# Autodesk Inventor assembly: アーム ツインロッドアーム先端アセンブリ
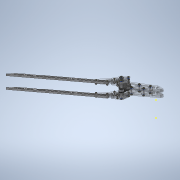
[picture p0: Inventor's stored thumbnail of the model, 180x180]
Saved by Autodesk Inventor 2020.2 (Build 242310000, 310)
## iProperties
Created: 2018-11-26
Part Number: アーム ツインロッドアーム先端アセンブリ
Material: 一般
Document SubType Name: Assembly
Designer: 雪村
Mass: 174.621 g
Surface Area: 858.198 cm^2
Volume: 87.2019 cm^3
Density: 2.00249 g/cm^3
Author: 雪村
## Documents named in this file (16)
- C:\Users\mozar\Desktop\院2年機大型\アーム ツインロッドアーム先端アセンブリ.iam
- C:\Users\mozar\Desktop\院2年機大型\アーム アーム先端根本ポリカパーツ.ipt
- C:\Users\mozar\Desktop\院2年機大型\アーム アーム先端根本ポリカパーツ(ミラー).ipt
- C:\Users\mozar\Desktop\院2年機大型\既製品\スペーサーm3-16　簡易筒型.ipt
- C:\Users\mozar\Desktop\院2年機大型\アーム ツインアーム先端押さえ.ipt
- C:\Users\mozar\Desktop\院2年機大型\既製品\ねじ\SB　M4 8mm なべネジ.ipt
- C:\Users\mozar\Desktop\院2年機大型\既製品\セットカラー　内径6.ipt
- C:\Users\mozar\Desktop\院2年機大型\アーム 中間節 先端中詰め.ipt
- C:\Users\mozar\Desktop\院2年機大型\既製品\スペーサーm3-60　簡易筒型　売ってない.ipt
- C:\Users\mozar\Desktop\院2年機大型\既製品\ねじ\SB　6mmなべネジ.ipt
- C:\Users\mozar\Desktop\院2年機大型\既製品\ねじ\ナイロンナットm3.ipt
- C:\Users\mozar\Desktop\院2年機大型\アーム アーム先端長め丹治type.ipt
- C:\Users\mozar\Desktop\院2年機大型\アーム ツインアーム先端 ポリカフリー部5t(ミラー).ipt
- C:\Users\mozar\Desktop\院2年機大型\アーム ツインアーム先端 ポリカフリー部5t.ipt
- C:\Users\mozar\Desktop\院2年機大型\既製品\オイレス　6-8-12　フランジ付き　（L=5）.ipt
- C:\Users\mozar\Desktop\院2年機大型\既製品\ねじ\SB　14mmなべネジ.ipt
## Components (60 placed, 15 different names)
1. アーム アーム先端根本ポリカパーツ:1 — 挿入:230, 挿入:231, 挿入:232, 挿入:233, 挿入:250, 挿入:251, 挿入:252, 挿入:253, メイト:10
2. アーム アーム先端根本ポリカパーツ(ミラー):1 — 挿入:246, 挿入:247, 挿入:248, 挿入:249, 挿入:259, メイト:8, メイト:9, 挿入:294
3. アーム ツインアーム先端押さえ:1 — 挿入:265, 挿入:266, 挿入:268, 挿入:269, 挿入:270
4. アーム ツインアーム先端押さえ:2 — 挿入:260, 挿入:261, 挿入:262, 挿入:271, 挿入:272, 挿入:273
5. スペーサーm3-16　簡易筒型:4 — 挿入:230
6. スペーサーm3-16　簡易筒型:5 — 挿入:231, 挿入:294
7. スペーサーm3-16　簡易筒型:6 — 挿入:232
8. スペーサーm3-16　簡易筒型:7 — 挿入:233
9. SB　M4 8mm なべネジ:6 — 挿入:248
10. SB　M4 8mm なべネジ:8 — 挿入:249
11. SB　M4 8mm なべネジ:9 — 挿入:252
12. SB　M4 8mm なべネジ:14 — 挿入:246
13. SB　M4 8mm なべネジ:17 — 挿入:247
14. SB　M4 8mm なべネジ:18 — 挿入:250
15. SB　M4 8mm なべネジ:19 — 挿入:251
16. SB　M4 8mm なべネジ:20 — 挿入:253
17. セットカラー　内径6:3 — 挿入:255
18. セットカラー　内径6:4 — 挿入:254, 挿入:257
19. セットカラー　内径6:5 — 挿入:256, 挿入:258
20. アーム 中間節 先端中詰め:1 — 挿入:254, 挿入:255, 挿入:256
21. アーム 中間節 先端中詰め:2 — 挿入:257, 挿入:258, 挿入:259, メイト:8
22. スペーサーm3-60　簡易筒型　売ってない:1 — 挿入:260, メイト:9, 挿入:266, メイト:10
23. スペーサーm3-60　簡易筒型　売ってない:2 — 挿入:261, 挿入:265, 挿入:307, 挿入:308
24. スペーサーm3-60　簡易筒型　売ってない:3 — 挿入:262
25. SB　6mmなべネジ:1 — 挿入:268
26. SB　6mmなべネジ:2 — 挿入:270
27. SB　6mmなべネジ:3 — 挿入:269
28. SB　6mmなべネジ:4 — 挿入:273
29. SB　6mmなべネジ:5 — 挿入:272
30. SB　6mmなべネジ:6 — 挿入:271
31. ナイロンナットm3:1 — 挿入:326
32. ナイロンナットm3:5 — 挿入:324
33. ナイロンナットm3:12 — 挿入:327
34. ナイロンナットm3:13 — 挿入:320
35. ナイロンナットm3:14 — 挿入:325
36. ナイロンナットm3:16 — 挿入:319
37. ナイロンナットm3:17 — 挿入:328
38. アーム アーム先端長め丹治type:1 — 挿入:303, 挿入:304
39. アーム アーム先端長め丹治type:2 — 挿入:305, 挿入:306
40. アーム ツインアーム先端 ポリカフリー部5t(ミラー):1 — 挿入:296, 挿入:299, 挿入:300, 挿入:314, 挿入:315, 挿入:316, 挿入:317, 挿入:318
41. アーム ツインアーム先端 ポリカフリー部5t:1 — 挿入:295, 挿入:299, 挿入:300, 挿入:303, 挿入:304, 挿入:319, 挿入:320, 挿入:321, 挿入:322, 挿入:323
42. アーム ツインアーム先端 ポリカフリー部5t(ミラー):2 — 挿入:297, 挿入:301, 挿入:302, 挿入:324, 挿入:325, 挿入:326, 挿入:327, 挿入:328
43. アーム ツインアーム先端 ポリカフリー部5t:2 — 挿入:298, 挿入:301, 挿入:302, 挿入:305, 挿入:306, 挿入:309, 挿入:310, 挿入:311, 挿入:312, 挿入:313
44. オイレス　6-8-12　フランジ付き　（L=5）:1 — 挿入:297
45. オイレス　6-8-12　フランジ付き　（L=5）:2 — 挿入:298, 挿入:308
46. オイレス　6-8-12　フランジ付き　（L=5）:3 — 挿入:296, 挿入:307
47. オイレス　6-8-12　フランジ付き　（L=5）:4 — 挿入:295
48. SB　14mmなべネジ:1 — 挿入:310
49. SB　14mmなべネジ:2 — 挿入:311
50. SB　14mmなべネジ:3 — 挿入:309
51. SB　14mmなべネジ:4 — 挿入:312
52. SB　14mmなべネジ:5 — 挿入:318
53. SB　14mmなべネジ:6 — 挿入:316
54. SB　14mmなべネジ:7 — 挿入:315
55. SB　14mmなべネジ:8 — 挿入:317
56. SB　14mmなべネジ:9 — 挿入:314
57. SB　14mmなべネジ:10 — 挿入:313
58. ナイロンナットm3:18 — 挿入:321
59. ナイロンナットm3:19 — 挿入:322
60. ナイロンナットm3:20 — 挿入:323
## Relationships (67: Insert 64, Mate 3)
- 挿入:230 [Insert]: アーム アーム先端根本ポリカパーツ:1 ↔ スペーサーm3-16　簡易筒型:4
- 挿入:231 [Insert]: アーム アーム先端根本ポリカパーツ:1 ↔ スペーサーm3-16　簡易筒型:5
- 挿入:232 [Insert]: アーム アーム先端根本ポリカパーツ:1 ↔ スペーサーm3-16　簡易筒型:6
- 挿入:233 [Insert]: アーム アーム先端根本ポリカパーツ:1 ↔ スペーサーm3-16　簡易筒型:7
- 挿入:246 [Insert]: アーム アーム先端根本ポリカパーツ(ミラー):1 ↔ SB　M4 8mm なべネジ:14
- 挿入:247 [Insert]: アーム アーム先端根本ポリカパーツ(ミラー):1 ↔ SB　M4 8mm なべネジ:17
- 挿入:248 [Insert]: アーム アーム先端根本ポリカパーツ(ミラー):1 ↔ SB　M4 8mm なべネジ:6
- 挿入:249 [Insert]: アーム アーム先端根本ポリカパーツ(ミラー):1 ↔ SB　M4 8mm なべネジ:8
- 挿入:250 [Insert]: アーム アーム先端根本ポリカパーツ:1 ↔ SB　M4 8mm なべネジ:18
- 挿入:251 [Insert]: アーム アーム先端根本ポリカパーツ:1 ↔ SB　M4 8mm なべネジ:19
- 挿入:252 [Insert]: アーム アーム先端根本ポリカパーツ:1 ↔ SB　M4 8mm なべネジ:9
- 挿入:253 [Insert]: アーム アーム先端根本ポリカパーツ:1 ↔ SB　M4 8mm なべネジ:20
- 挿入:254 [Insert]: セットカラー　内径6:4 ↔ アーム 中間節 先端中詰め:1
- 挿入:255 [Insert]: セットカラー　内径6:3 ↔ アーム 中間節 先端中詰め:1
- 挿入:256 [Insert]: セットカラー　内径6:5 ↔ アーム 中間節 先端中詰め:1
- 挿入:257 [Insert]: セットカラー　内径6:4 ↔ アーム 中間節 先端中詰め:2
- 挿入:258 [Insert]: セットカラー　内径6:5 ↔ アーム 中間節 先端中詰め:2
- 挿入:259 [Insert]: アーム アーム先端根本ポリカパーツ(ミラー):1 ↔ アーム 中間節 先端中詰め:2
- メイト:8 [Mate]: アーム アーム先端根本ポリカパーツ(ミラー):1 ↔ アーム 中間節 先端中詰め:2
- 挿入:260 [Insert]: アーム ツインアーム先端押さえ:2 ↔ スペーサーm3-60　簡易筒型　売ってない:1
- 挿入:261 [Insert]: アーム ツインアーム先端押さえ:2 ↔ スペーサーm3-60　簡易筒型　売ってない:2
- 挿入:262 [Insert]: アーム ツインアーム先端押さえ:2 ↔ スペーサーm3-60　簡易筒型　売ってない:3
- メイト:9 [Mate]: アーム アーム先端根本ポリカパーツ(ミラー):1 ↔ スペーサーm3-60　簡易筒型　売ってない:1
- 挿入:265 [Insert]: アーム ツインアーム先端押さえ:1 ↔ スペーサーm3-60　簡易筒型　売ってない:2
- 挿入:266 [Insert]: アーム ツインアーム先端押さえ:1 ↔ スペーサーm3-60　簡易筒型　売ってない:1
- 挿入:268 [Insert]: アーム ツインアーム先端押さえ:1 ↔ SB　6mmなべネジ:1
- 挿入:269 [Insert]: アーム ツインアーム先端押さえ:1 ↔ SB　6mmなべネジ:3
- 挿入:270 [Insert]: アーム ツインアーム先端押さえ:1 ↔ SB　6mmなべネジ:2
- 挿入:271 [Insert]: アーム ツインアーム先端押さえ:2 ↔ SB　6mmなべネジ:6
- 挿入:272 [Insert]: アーム ツインアーム先端押さえ:2 ↔ SB　6mmなべネジ:5
- 挿入:273 [Insert]: アーム ツインアーム先端押さえ:2 ↔ SB　6mmなべネジ:4
- メイト:10 [Mate]: アーム アーム先端根本ポリカパーツ:1 ↔ スペーサーm3-60　簡易筒型　売ってない:1
- 挿入:294 [Insert]: アーム アーム先端根本ポリカパーツ(ミラー):1 ↔ スペーサーm3-16　簡易筒型:5
- 挿入:295 [Insert]: アーム ツインアーム先端 ポリカフリー部5t:1 ↔ オイレス　6-8-12　フランジ付き　（L=5）:4
- 挿入:296 [Insert]: アーム ツインアーム先端 ポリカフリー部5t(ミラー):1 ↔ オイレス　6-8-12　フランジ付き　（L=5）:3
- 挿入:297 [Insert]: アーム ツインアーム先端 ポリカフリー部5t(ミラー):2 ↔ オイレス　6-8-12　フランジ付き　（L=5）:1
- 挿入:298 [Insert]: アーム ツインアーム先端 ポリカフリー部5t:2 ↔ オイレス　6-8-12　フランジ付き　（L=5）:2
- 挿入:299 [Insert]: アーム ツインアーム先端 ポリカフリー部5t(ミラー):1 ↔ アーム ツインアーム先端 ポリカフリー部5t:1
- 挿入:300 [Insert]: アーム ツインアーム先端 ポリカフリー部5t(ミラー):1 ↔ アーム ツインアーム先端 ポリカフリー部5t:1
- 挿入:301 [Insert]: アーム ツインアーム先端 ポリカフリー部5t(ミラー):2 ↔ アーム ツインアーム先端 ポリカフリー部5t:2
- 挿入:302 [Insert]: アーム ツインアーム先端 ポリカフリー部5t(ミラー):2 ↔ アーム ツインアーム先端 ポリカフリー部5t:2
- 挿入:303 [Insert]: アーム アーム先端長め丹治type:1 ↔ アーム ツインアーム先端 ポリカフリー部5t:1
- 挿入:304 [Insert]: アーム アーム先端長め丹治type:1 ↔ アーム ツインアーム先端 ポリカフリー部5t:1
- 挿入:305 [Insert]: アーム アーム先端長め丹治type:2 ↔ アーム ツインアーム先端 ポリカフリー部5t:2
- 挿入:306 [Insert]: アーム アーム先端長め丹治type:2 ↔ アーム ツインアーム先端 ポリカフリー部5t:2
- 挿入:307 [Insert]: スペーサーm3-60　簡易筒型　売ってない:2 ↔ オイレス　6-8-12　フランジ付き　（L=5）:3
- 挿入:308 [Insert]: スペーサーm3-60　簡易筒型　売ってない:2 ↔ オイレス　6-8-12　フランジ付き　（L=5）:2
- 挿入:309 [Insert]: アーム ツインアーム先端 ポリカフリー部5t:2 ↔ SB　14mmなべネジ:3
- 挿入:310 [Insert]: アーム ツインアーム先端 ポリカフリー部5t:2 ↔ SB　14mmなべネジ:1
- 挿入:311 [Insert]: アーム ツインアーム先端 ポリカフリー部5t:2 ↔ SB　14mmなべネジ:2
- 挿入:312 [Insert]: アーム ツインアーム先端 ポリカフリー部5t:2 ↔ SB　14mmなべネジ:4
- 挿入:313 [Insert]: アーム ツインアーム先端 ポリカフリー部5t:2 ↔ SB　14mmなべネジ:10
- 挿入:314 [Insert]: アーム ツインアーム先端 ポリカフリー部5t(ミラー):1 ↔ SB　14mmなべネジ:9
- 挿入:315 [Insert]: アーム ツインアーム先端 ポリカフリー部5t(ミラー):1 ↔ SB　14mmなべネジ:7
- 挿入:316 [Insert]: アーム ツインアーム先端 ポリカフリー部5t(ミラー):1 ↔ SB　14mmなべネジ:6
- 挿入:317 [Insert]: アーム ツインアーム先端 ポリカフリー部5t(ミラー):1 ↔ SB　14mmなべネジ:8
- 挿入:318 [Insert]: アーム ツインアーム先端 ポリカフリー部5t(ミラー):1 ↔ SB　14mmなべネジ:5
- 挿入:319 [Insert]: ナイロンナットm3:16 ↔ アーム ツインアーム先端 ポリカフリー部5t:1
- 挿入:320 [Insert]: ナイロンナットm3:13 ↔ アーム ツインアーム先端 ポリカフリー部5t:1
- 挿入:321 [Insert]: アーム ツインアーム先端 ポリカフリー部5t:1 ↔ ナイロンナットm3:18
- 挿入:322 [Insert]: アーム ツインアーム先端 ポリカフリー部5t:1 ↔ ナイロンナットm3:19
- 挿入:323 [Insert]: アーム ツインアーム先端 ポリカフリー部5t:1 ↔ ナイロンナットm3:20
- 挿入:324 [Insert]: ナイロンナットm3:5 ↔ アーム ツインアーム先端 ポリカフリー部5t(ミラー):2
- 挿入:325 [Insert]: ナイロンナットm3:14 ↔ アーム ツインアーム先端 ポリカフリー部5t(ミラー):2
- 挿入:326 [Insert]: ナイロンナットm3:1 ↔ アーム ツインアーム先端 ポリカフリー部5t(ミラー):2
- 挿入:327 [Insert]: ナイロンナットm3:12 ↔ アーム ツインアーム先端 ポリカフリー部5t(ミラー):2
- 挿入:328 [Insert]: ナイロンナットm3:17 ↔ アーム ツインアーム先端 ポリカフリー部5t(ミラー):2
